# Autodesk Inventor assembly: Body Assembly
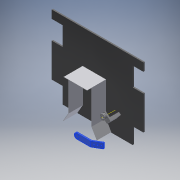
[picture p0: Inventor's stored thumbnail of the model, 180x180]
Saved by Autodesk Inventor 2019 (Build 230136000, 136)
## iProperties
Created: 2019-10-15
Part Number: Body Assembly
Document SubType Name: Assembly
Designer: User
Author: User
## Documents named in this file (6)
- C:\Robotics\CAD\2019-20_CAD\Collection\Body Assembly.iam
- C:\Robotics\CAD\2019-20_CAD\Collection\U-Part Gen 2.ipt
- C:\Robotics\CAD\COTSParts\Actobotics\545 parts\545364 assembly.ipt
- C:\Robotics\CAD\2019-20_CAD\Collection\wheel arm stand off.ipt
- C:\Robotics\CAD\2019-20_CAD\Drive Train\Gen 2.0 rev mecanums base plate.ipt
- C:\Robotics\CAD\2019-20_CAD\Collection\arm assembaly.iam
## Components (5 placed, 5 different names)
1. U-Part Gen 2:1 — Mate:19, Flush:8
2. 545364 assembly:2 — Mate:17, Mate:18, Mate:20
3. wheel arm stand off:2 — Mate:17, Mate:18
4. Gen 2.0 rev mecanums base plate:1 — Mate:19, Flush:8
5. arm assembaly:1 [sub-assembly] — Mate:20
## Relationships (5: Mate 4, Flush 1)
- Mate:17: 545364 assembly:2 ↔ wheel arm stand off:2
- Mate:18: 545364 assembly:2 ↔ wheel arm stand off:2
- Mate:19: U-Part Gen 2:1 ↔ Gen 2.0 rev mecanums base plate:1
- Flush:8 (203.2 mm): U-Part Gen 2:1 ↔ Gen 2.0 rev mecanums base plate:1
- Mate:20: 545364 assembly:2 ↔ arm assembaly:1
